# Autodesk Inventor assembly: Assembly3
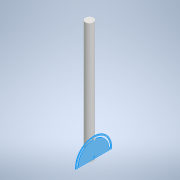
[picture p0: Inventor's stored thumbnail of the model, 180x180]
Saved by Autodesk Inventor 2020.2 (Build 242310000, 310)
## iProperties
Created: 2020-02-19
Part Number: Assembly3
Document SubType Name: Assembly
Designer: lenovo
Author: lenovo
## Documents named in this file (3)
- D:\BE II Year\eng exploration\notes\Assembly3.iam
- D:\BE II Year\eng exploration\notes\trail 12.ipt
- D:\BE II Year\eng exploration\notes\trail 9.ipt
## Components (2 placed, 2 different names)
1. trail 12:1 — Rigid:1
2. trail 9:1 — Rigid:1
## Relationships (1: WeldJoint 1)
- Rigid:1 [WeldJoint] (1 mm): trail 12:1 ↔ trail 9:1
